# Autodesk Inventor assembly: 2f1
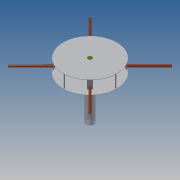
[picture p0: Inventor's stored thumbnail of the model, 180x180]
Saved by Autodesk Inventor 2014 SP1 (Build 180222100, 222)
## iProperties
Created: 2013-05-22
Part Number: 2f1
Document SubType Name: Assembly
Designer: Dave
Description: Feed dipole
Author: Dave
## Documents named in this file (10)
- C:\Users\Dave\Desktop\hera-cad\feed\dipole.iam
- C:\Users\Dave\Desktop\hera-cad\feed\dipoleBottomDisc.ipt
- C:\Users\Dave\Desktop\hera-cad\feed\dipoleArm.ipt
- C:\Users\Dave\Desktop\hera-cad\feed\dipoleDiscSpacer.ipt
- C:\Users\Dave\Desktop\hera-cad\feed\collar.ipt
- C:\Users\Dave\Desktop\hera-cad\feed\dipoleMast.ipt
- C:\Users\Dave\Desktop\hera-cad\feed\dipoleArmHold.ipt
- C:\Users\Dave\Desktop\hera-cad\feed\dipoleArmRest.ipt
- C:\Users\Dave\Desktop\hera-cad\feed\dipoleTopDisc.ipt
- C:\Users\Dave\Desktop\hera-cad\feed\matingBoard.ipt
## Components (21 placed, 9 different names)
1. dipoleBottomDisc:1 — Insert:5, Insert:8, Insert:9, Insert:12, Insert:13, Insert:18, Insert:19, Insert:20
2. dipoleDiscSpacer:2 — Insert:5, Insert:21
3. dipoleDiscSpacer:3 — Insert:18, Insert:22
4. dipoleDiscSpacer:4 — Insert:19
5. dipoleDiscSpacer:5 — Insert:20
6. dipoleTopDisc:1 — Insert:16, Insert:17, Insert:21, Insert:22, Insert:23
7. matingBoard:1 — Insert:10, Insert:11, Insert:12, Insert:13
8. collar:1 — Insert:16, Insert:17
9. dipoleMast:1 — Insert:23
10. dipoleArmHold:1 — Insert:4, Insert:8, Insert:9
11. dipoleArm:1 — Insert:4
12. dipoleArmRest:1 — Insert:10, Insert:11
13. dipoleArmHold:2
14. dipoleArm:2
15. dipoleArmRest:2
16. dipoleArmHold:3
17. dipoleArm:3
18. dipoleArmRest:3
19. dipoleArmHold:4
20. dipoleArm:4
21. dipoleArmRest:4
## Component patterns: arms (4 elements)
## Relationships (16: Insert 16)
- Insert:4 (-275.59 mm): dipoleArmHold:1 ↔ dipoleArm:1
- Insert:5: dipoleBottomDisc:1 ↔ dipoleDiscSpacer:2
- Insert:8: dipoleBottomDisc:1 ↔ dipoleArmHold:1
- Insert:9: dipoleBottomDisc:1 ↔ dipoleArmHold:1
- Insert:10: matingBoard:1 ↔ dipoleArmRest:1
- Insert:11: matingBoard:1 ↔ dipoleArmRest:1
- Insert:12: dipoleBottomDisc:1 ↔ matingBoard:1
- Insert:13: dipoleBottomDisc:1 ↔ matingBoard:1
- Insert:16: dipoleTopDisc:1 ↔ collar:1
- Insert:17: dipoleTopDisc:1 ↔ collar:1
- Insert:18: dipoleBottomDisc:1 ↔ dipoleDiscSpacer:3
- Insert:19: dipoleBottomDisc:1 ↔ dipoleDiscSpacer:4
- Insert:20: dipoleBottomDisc:1 ↔ dipoleDiscSpacer:5
- Insert:21: dipoleDiscSpacer:2 ↔ dipoleTopDisc:1
- Insert:22: dipoleDiscSpacer:3 ↔ dipoleTopDisc:1
- Insert:23: dipoleTopDisc:1 ↔ dipoleMast:1
